# Autodesk Inventor assembly: Assembly1
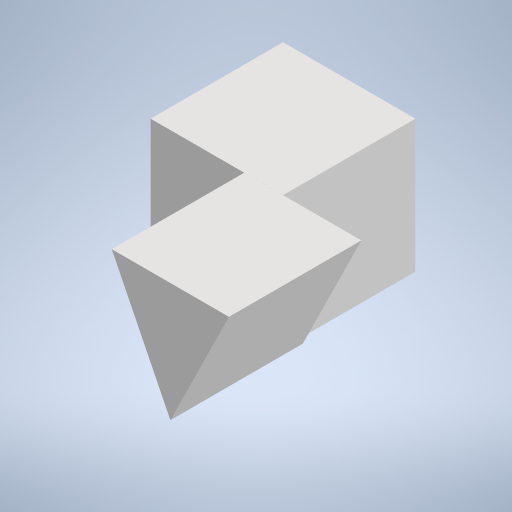
[picture p0: Inventor's stored thumbnail of the model, 512x512]
Saved by Autodesk Inventor 2023.1 (Build 271208000, 208)
## iProperties
Created: 2022-08-11
Part Number: Assembly1
Document SubType Name: Assembly
Designer: Robotics
Author: Robotics
## Documents named in this file (3)
- W:\2022-2023 Season\2022 Offseason\Assembly1.iam
- W:\2022-2023 Season\2022 Offseason\Part1.ipt
- W:\2022-2023 Season\2022 Offseason\Part2.ipt
## Components (2 placed, 2 different names)
1. Part1:1 — Mate:1, Flush:1
2. Part2:1 — Mate:1, Flush:1
## Relationships (2: Mate 1, Flush 1)
- Mate:1: Part1:1 ↔ Part2:1
- Flush:1: Part1:1 ↔ Part2:1
